# Autodesk Inventor assembly: EL2-C-100
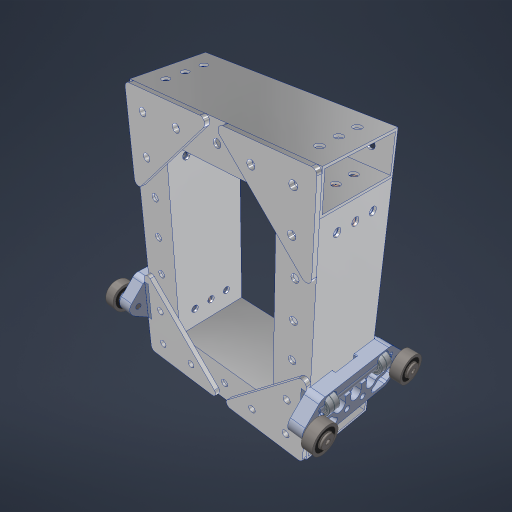
[picture p0: Inventor's stored thumbnail of the model, 512x512]
Saved by Autodesk Inventor 2023.4 (Build 274418000, 418)
## iProperties
Created: 2025-01-11
Part Number: EL2-C-100
Document SubType Name: Assembly
Designer: brand
Author: brand
## Documents named in this file (5)
- C:\Users\brand\OneDrive\Documents\GitHub\robotics 23\2025-ReefScape---CAD\Elevator\EL2\EL2-C-100.iam
- C:\Users\brand\OneDrive\Documents\GitHub\robotics 23\2025-ReefScape---CAD\Elevator\EL2\EL2-C-001.ipt
- C:\Users\brand\OneDrive\Documents\GitHub\robotics 23\2025-ReefScape---CAD\COMMON PARTS\WCP Elevator parts\WCP-0897\WCP-0897.iam
- C:\Users\brand\OneDrive\Documents\GitHub\robotics 23\2025-ReefScape---CAD\Elevator\EL2\EL2-005.ipt
- C:\Users\brand\OneDrive\Documents\GitHub\robotics 23\2025-ReefScape---CAD\Elevator\EL2\EL2-C-002.ipt
## Components (14 placed, 4 different names)
1. EL2-C-001:1 — Insert:5, Insert:7, Insert:11, Insert:13
2. EL2-C-001:2 — Insert:1, Angle:1, Insert:2, Angle:2, Insert:3, Insert:4, Insert:6, Insert:16, Angle:5
3. EL2-C-001:3 — Insert:8, Angle:3, Insert:9, Insert:10, Angle:4, Insert:12, Insert:18
4. EL2-C-001:4 — Insert:14, Insert:15, Insert:17, Insert:19
5. WCP-0897:1 [sub-assembly] — Insert:9
6. WCP-0897:2 [sub-assembly] — Insert:3, Insert:4
7. EL2-005:1 — Insert:2, Angle:2
8. EL2-005:2 — Insert:8, Angle:3
9. EL2-005:3 — Insert:10, Angle:4
10. EL2-005:4 — Insert:1, Angle:1
11. EL2-C-002:1 — Insert:5, Insert:6, Insert:7, Angle:5
12. EL2-C-002:2 — Insert:11, Insert:12, Insert:13
13. EL2-C-002:3 — Insert:17, Insert:18, Insert:19
14. EL2-C-002:4 — Insert:14, Insert:15, Insert:16
## Relationships (24: Insert 19, Angle 5)
- Insert:1: EL2-C-001:2 ↔ EL2-005:4
- Angle:1 (0 deg): EL2-C-001:2 ↔ EL2-005:4
- Insert:2: EL2-C-001:2 ↔ EL2-005:1
- Angle:2 (0 deg): EL2-C-001:2 ↔ EL2-005:1
- Insert:3: EL2-C-001:2 ↔ WCP-0897:2
- Insert:4: EL2-C-001:2 ↔ WCP-0897:2
- Insert:5: EL2-C-001:1 ↔ EL2-C-002:1
- Insert:6: EL2-C-001:2 ↔ EL2-C-002:1
- Insert:7: EL2-C-001:1 ↔ EL2-C-002:1
- Insert:8: EL2-C-001:3 ↔ EL2-005:2
- Angle:3 (0 deg): EL2-C-001:3 ↔ EL2-005:2
- Insert:9: EL2-C-001:3 ↔ WCP-0897:1
- Insert:10: EL2-C-001:3 ↔ EL2-005:3
- Angle:4 (0 deg): EL2-C-001:3 ↔ EL2-005:3
- Insert:11: EL2-C-001:1 ↔ EL2-C-002:2
- Insert:12: EL2-C-001:3 ↔ EL2-C-002:2
- Insert:13: EL2-C-001:1 ↔ EL2-C-002:2
- Insert:14: EL2-C-001:4 ↔ EL2-C-002:4
- Insert:15: EL2-C-001:4 ↔ EL2-C-002:4
- Insert:16: EL2-C-001:2 ↔ EL2-C-002:4
- Insert:17: EL2-C-001:4 ↔ EL2-C-002:3
- Insert:18: EL2-C-001:3 ↔ EL2-C-002:3
- Insert:19: EL2-C-001:4 ↔ EL2-C-002:3
- Angle:5 (0 deg): EL2-C-001:2 ↔ EL2-C-002:1
